# Autodesk Inventor assembly: A_MiniDrone
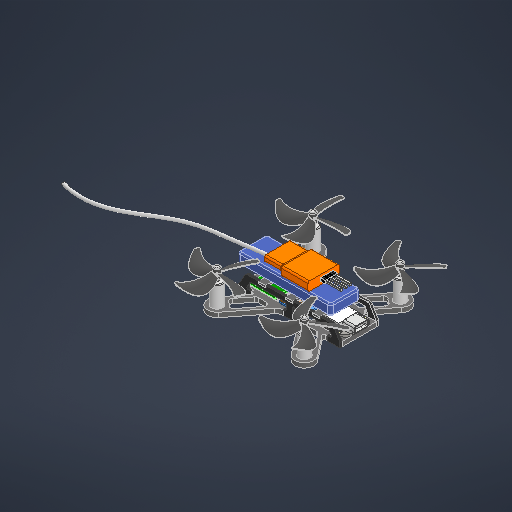
[picture p0: Inventor's stored thumbnail of the model, 512x512]
Saved by Autodesk Inventor 2026.2 (Build 302298000, 298)
## iProperties
Created: 2026-02-08
Part Number: A_MiniDrone
Document SubType Name: Assembly
Designer: FAL
Author: FAL
## Documents named in this file (12)
- C:\Users\FAL\git\ESP32-Drone\Hardware\CAD\V4\A_MiniDrone.iam
- C:\Users\FAL\git\ESP32-Drone\Hardware\CAD\V4\P_Motor.ipt
- C:\Users\FAL\git\ESP32-Drone\Hardware\CAD\V4\P_DroneCase.ipt
- C:\Users\FAL\projects\_libary\electronic\microcontroller\esp32\esp32-C3\ESP32-C3_SEEED\ESP32-C3_SEEED\ESP32-C3_SEEED.ipt
- C:\Users\FAL\git\ESP32-Drone\Hardware\CAD\V4\P_Akku_1S.ipt
- C:\Users\FAL\git\ESP32-Drone\Hardware\CAD\V4\P_Prop_4_blade.ipt
- C:\Users\FAL\git\ESP32-Drone\Hardware\CAD\V4\P_R6DSM.ipt
- C:\Users\FAL\projects\_libary\electronic\sensors\MPU6050\MPU6050 v2\MPU6050 v2\MPU6050 v2.ipt
- C:\Users\FAL\git\sim_stick\Hardware\P_driver.ipt
- C:\Users\FAL\git\sim_stick\Hardware\P_Side.ipt
- C:\Users\FAL\git\sim_stick\Hardware\P_board.ipt
- C:\Users\FAL\git\sim_stick\Hardware\P_Side_MIR.ipt
## Components (19 placed, 11 different names)
1. P_Motor:1 — Passend:10, Fluchtend:7, Fluchtend:8, Fluchtend:9, Fluchtend:11, Passend:36
2. P_Motor:2 — Passend:1, Passend:12, Fluchtend:5, Passend:20
3. P_Motor:3 — Passend:9, Fluchtend:4, Passend:17, Fluchtend:9
4. P_Motor:4 — Passend:11, Fluchtend:6, Passend:19, Fluchtend:8, Passend:20
5. P_DroneCase:1 — Fluchtend:1, Fluchtend:2, Fluchtend:3, Passend:1, Passend:17, Passend:19, Fluchtend:11, Passend:25, Passend:35, Passend:36, Fluchtend:17
6. ESP32-C3_SEEED:1 — Passend:8, Passend:35, Fluchtend:17
7. P_Akku_1S:1 — Passend:6, Passend:34
8. P_Prop_4_blade:1 — Passend:9, Fluchtend:4
9. P_Prop_4_blade:2 — Passend:12, Fluchtend:5
10. P_Prop_4_blade:3 — Passend:10, Fluchtend:7
11. P_Prop_4_blade:4 — Passend:11, Fluchtend:6
12. P_R6DSM:1 — Fluchtend:16
13. MPU6050 v2:1 — Passend:21
14. P_driver:1 — Passend:22, Passend:25
15. P_Side:1 — Passend:23, Passend:24, Fluchtend:10, Fluchtend:12, Passend:26, Passend:27, Passend:28, Fluchtend:13, Passend:29, Fluchtend:14, Passend:30, Passend:31
16. P_board:1 — Fluchtend:12, Passend:26, Passend:27
17. P_board:2 — Fluchtend:14, Passend:30, Passend:31
18. P_board:3 — Passend:28, Fluchtend:13, Passend:29, Passend:34
19. P_Side_MIR:1 — Passend:32, Fluchtend:15, Passend:33
## Relationships (43: Mate 26, Flush 17)
- Fluchtend:1 [Flush]: P_DroneCase:1
- Fluchtend:2 [Flush]: P_DroneCase:1
- Fluchtend:3 [Flush]: P_DroneCase:1
- Passend:1 [Mate]: P_Motor:2 ↔ P_DroneCase:1
- Passend:6 [Mate]: P_Akku_1S:1
- Passend:8 [Mate]: ESP32-C3_SEEED:1
- Passend:9 [Mate]: P_Motor:3 ↔ P_Prop_4_blade:1
- Fluchtend:4 [Flush]: P_Motor:3 ↔ P_Prop_4_blade:1
- Passend:10 [Mate]: P_Motor:1 ↔ P_Prop_4_blade:3
- Passend:11 [Mate]: P_Motor:4 ↔ P_Prop_4_blade:4
- Passend:12 [Mate]: P_Motor:2 ↔ P_Prop_4_blade:2
- Fluchtend:5 [Flush]: P_Motor:2 ↔ P_Prop_4_blade:2
- Fluchtend:6 [Flush]: P_Motor:4 ↔ P_Prop_4_blade:4
- Fluchtend:7 [Flush]: P_Motor:1 ↔ P_Prop_4_blade:3
- Passend:17 [Mate]: P_Motor:3 ↔ P_DroneCase:1
- Passend:19 [Mate]: P_Motor:4 ↔ P_DroneCase:1
- Fluchtend:8 [Flush]: P_Motor:1 ↔ P_Motor:4
- Fluchtend:9 [Flush]: P_Motor:1 ↔ P_Motor:3
- Passend:20 [Mate]: P_Motor:2 ↔ P_Motor:4
- Passend:21 [Mate]: MPU6050 v2:1
- Passend:22 [Mate]: P_driver:1
- Passend:23 [Mate]: P_Side:1
- Passend:24 [Mate]: P_Side:1
- Fluchtend:10 [Flush]: P_Side:1
- Fluchtend:11 [Flush]: P_Motor:1 ↔ P_DroneCase:1
- Passend:25 [Mate]: P_DroneCase:1 ↔ P_driver:1
- Fluchtend:12 [Flush]: P_Side:1 ↔ P_board:1
- Passend:26 [Mate]: P_Side:1 ↔ P_board:1
- Passend:27 [Mate]: P_Side:1 ↔ P_board:1
- Passend:28 [Mate]: P_Side:1 ↔ P_board:3
- Fluchtend:13 [Flush]: P_Side:1 ↔ P_board:3
- Passend:29 [Mate]: P_Side:1 ↔ P_board:3
- Fluchtend:14 [Flush]: P_Side:1 ↔ P_board:2
- Passend:30 [Mate]: P_Side:1 ↔ P_board:2
- Passend:31 [Mate]: P_Side:1 ↔ P_board:2
- Passend:32 [Mate]: P_Side_MIR:1
- Fluchtend:15 [Flush]: P_Side_MIR:1
- Passend:33 [Mate]: P_Side_MIR:1
- Passend:34 [Mate]: P_Akku_1S:1 ↔ P_board:3
- Fluchtend:16 [Flush]: P_R6DSM:1
- Passend:35 [Mate]: P_DroneCase:1 ↔ ESP32-C3_SEEED:1
- Passend:36 [Mate]: P_Motor:1 ↔ P_DroneCase:1
- Fluchtend:17 [Flush]: P_DroneCase:1 ↔ ESP32-C3_SEEED:1
